# Autodesk Inventor assembly: Assembly1
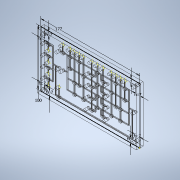
[picture p0: Inventor's stored thumbnail of the model, 180x180]
Saved by Autodesk Inventor 2021 (Build 250183000, 183)
## iProperties
Created: 2020-05-23
Part Number: Assembly1
Document SubType Name: Assembly
Designer: natha
Author: natha
## Documents named in this file (3)
- C:\03_Dokumente\02_Master_Uni_Stuttgart\06_Studienarbeit Ausland\02_Work\04_CAD\First Board\Millifluidic Board.iam
- C:\03_Dokumente\02_Master_Uni_Stuttgart\06_Studienarbeit Ausland\02_Work\04_CAD\First Board\Flow Layer.ipt
- C:\03_Dokumente\02_Master_Uni_Stuttgart\06_Studienarbeit Ausland\02_Work\04_CAD\First Board\Control Layer.ipt
## Components (2 placed, 2 different names)
1. Flow Layer:1 — Mate:1
2. Control Layer:1 — Mate:2
## Relationships (2: Mate 2)
- Mate:1: Flow Layer:1
- Mate:2: Control Layer:1
